# Autodesk Inventor assembly: MainModule
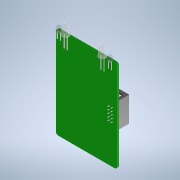
[picture p0: Inventor's stored thumbnail of the model, 180x180]
Saved by Autodesk Inventor 2021 (Build 250183000, 183)
## iProperties
Created: 2021-05-14
Part Number: MainModule
Document SubType Name: Assembly
Designer: ermoz
Author: ermoz
## Documents named in this file (7)
- D:\Moje Wyczyny\My_Poor_Projects\Sneak100_MiniSumo\minisumo-sneak100\mechanics\ElectricElements\MainModule.iam
- D:\Moje Wyczyny\My_Poor_Projects\Sneak100_MiniSumo\minisumo-sneak100\mechanics\ElectricElements\MainBoard.ipt
- D:\Moje Wyczyny\My_Poor_Projects\Sneak100_MiniSumo\minisumo-sneak100\mechanics\PreMadeParts\IDC_10_pin_connector.ipt
- D:\Moje Wyczyny\My_Poor_Projects\Sneak100_MiniSumo\minisumo-sneak100\mechanics\PreMadeParts\TSOP4838.ipt
- D:\Moje Wyczyny\My_Poor_Projects\Sneak100_MiniSumo\minisumo-sneak100\mechanics\PreMadeParts\STM32F303RE_LQFP64.ipt
- D:\Moje Wyczyny\My_Poor_Projects\Sneak100_MiniSumo\minisumo-sneak100\mechanics\PreMadeParts\OPE5594A.ipt
- D:\Moje Wyczyny\My_Poor_Projects\Sneak100_MiniSumo\minisumo-sneak100\mechanics\PreMadeParts\TEFT4300.ipt
## Components (8 placed, 6 different names)
1. MainBoard:1 — Mate:1, Mate:3, Mate:7
2. IDC_10_pin_connector:1 — Mate:1
3. STM32F303RE_LQFP64:1 — Mate:3
4. TSOP4838:5 — Mate:7
5. OPE5594A:1 — Flush:1, Flush:2, Flush:3
6. OPE5594A:2 — Flush:1, Flush:2
7. TEFT4300:1 — Flush:3, Flush:4, Flush:5
8. TEFT4300:2 — Flush:4, Flush:5
## Relationships (8: Flush 5, Mate 3)
- Mate:1: MainBoard:1 ↔ IDC_10_pin_connector:1
- Mate:3: MainBoard:1 ↔ STM32F303RE_LQFP64:1
- Mate:7 (3 mm): MainBoard:1 ↔ TSOP4838:5
- Flush:1: OPE5594A:1 ↔ OPE5594A:2
- Flush:2: OPE5594A:1 ↔ OPE5594A:2
- Flush:3: OPE5594A:1 ↔ TEFT4300:1
- Flush:4: TEFT4300:1 ↔ TEFT4300:2
- Flush:5: TEFT4300:1 ↔ TEFT4300:2
